# Autodesk Inventor assembly: 밑판받침대조립품
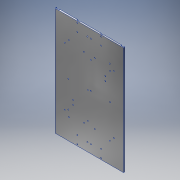
[picture p0: Inventor's stored thumbnail of the model, 180x180]
Saved by Autodesk Inventor 2017 (Build 210142000, 142)
## iProperties
Part Number: 밑판받침대조립품
Material: 일반
Document SubType Name: Assembly
Designer: minom
Mass: 360.826 g
Surface Area: 1853.85 cm^2
Volume: 133.639 cm^3
Density: 2.7 g/cm^3
Author: minom
## Documents named in this file (2)
- C:\Users\Minos\Documents\Inventor\Projects\2017 IRC Sumo Mino ver.2\밑판받침대조립품.iam
- C:\Users\Minos\Documents\Inventor\Projects\2017 IRC Sumo Mino ver.2\밑판_수정.ipt
## Components (1 placed, 1 different names)
1. 밑판_수정:1 — 메이트:1, 메이트:2
## Relationships (2: Mate 2)
- 메이트:1 [Mate] (10 mm): 밑판_수정:1
- 메이트:2 [Mate]: 밑판_수정:1
